# Autodesk Inventor assembly: Beamerscope_r2
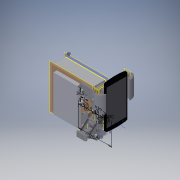
[picture p0: Inventor's stored thumbnail of the model, 180x180]
Saved by Autodesk Inventor 2016 (Build 200138000, 138)
## iProperties
Created: 2016-09-10
Part Number: Beamerscope_r2
Material: Generisch
Document SubType Name: Assembly
Designer: Bene
Mass: 220.683 g
Surface Area: 1737.49 cm^2
Volume: 289.423 cm^3
Density: 0.762493 g/cm^3
Author: Bene
## Documents named in this file (21)
- C:\Users\Bene\Dropbox\Dokumente\OpticalDesign\Beamerscope\Inventor\Beamerscope_r2\Beamerscope_r2.iam
- C:\Users\Bene\Dropbox\Dokumente\OpticalDesign\Beamerscope\Inventor\Beamerscope_r2\01_Beamer_Gehäuse.ipt
- C:\Users\Bene\Dropbox\Dokumente\OpticalDesign\Beamerscope\Inventor\Beamerscope_r2\02_Beamer_Deckel.ipt
- C:\Users\Bene\Dropbox\Dokumente\OpticalDesign\Beamerscope\Inventor\Beamerscope_r2\10_Mikrolinse.ipt
- C:\Users\Bene\Dropbox\Dokumente\OpticalDesign\Beamerscope\Inventor\Beamerscope_r2\11_Objektträger.ipt
- C:\Users\Bene\Dropbox\Dokumente\OpticalDesign\Beamerscope\Inventor\Beamerscope_r2\20_Z-Focus.ipt
- C:\Users\Bene\Dropbox\Dokumente\OpticalDesign\Beamerscope\Inventor\Beamerscope_r2\21_Connection_Projector_Focus.ipt
- C:\Users\Bene\Dropbox\Dokumente\OpticalDesign\Beamerscope\Inventor\Beamerscope_r2\31_Handyaufnahme_2.ipt
- C:\Users\Bene\Dropbox\Dokumente\OpticalDesign\Beamerscope\Inventor\Beamerscope_r2\31_Handyaufnahme_3.ipt
- C:\Users\Bene\Dropbox\Dokumente\OpticalDesign\Beamerscope\Inventor\Beamerscope_r2\00_SonyXperiaZ3correct.ipt
- C:\Users\Bene\Dropbox\Dokumente\OpticalDesign\Beamerscope\Inventor\Beamerscope_r2\32_Handycase.ipt
- C:\Users\Bene\Dropbox\Dokumente\OpticalDesign\Beamerscope\Inventor\Beamerscope_r2\22_Focus_Objectadapter.ipt
- C:\Users\Bene\Dropbox\Dokumente\OpticalDesign\Beamerscope\Inventor\Beamerscope_r2\31_Nexus 5.iam
- C:\Users\Bene\Dropbox\Dokumente\OpticalDesign\Beamerscope\Inventor\Beamerscope_r2\40_Adapter_Lens_Phone.ipt
- C:\Users\Bene\Dropbox\Dokumente\OpticalDesign\Beamerscope\Inventor\Beamerscope_r2\52_Bolzen.ipt
- C:\Users\Bene\Dropbox\Dokumente\OpticalDesign\Beamerscope\Inventor\Beamerscope_r2\22_Connection_Projector_Smartphone.ipt
- C:\Users\Bene\Dropbox\Dokumente\OpticalDesign\Beamerscope\Inventor\Beamerscope_r2\23_Connection_Smartphone.ipt
- C:\Users\Bene\Dropbox\Dokumente\OpticalDesign\Beamerscope\Inventor\Beamerscope_r2\00_Stange.ipt
- C:\Users\Bene\Dropbox\Dokumente\OpticalDesign\Beamerscope\Inventor\Beamerscope_r2\24_Klammer_rechts.ipt
- C:\Users\Bene\Dropbox\Dokumente\OpticalDesign\Beamerscope\Inventor\Beamerscope_r2\24_Klammer_links.ipt
- C:\Users\Bene\Dropbox\Dokumente\OpticalDesign\Beamerscope\Inventor\Beamerscope_r2\12_Lenstube.ipt
## Components (21 placed, 20 different names)
1. 01_Beamer_Gehäuse:1 — Fluchtend:1, Fluchtend:7, Fluchtend:8, Passend:6, Passend:7, Passend:8, Fluchtend:12, Fluchtend:13, Fluchtend:15, Fluchtend:24, Fluchtend:25, Passend:12
2. 02_Beamer_Deckel:1 — Fluchtend:1, Fluchtend:22
3. 10_Mikrolinse:1 — Passend:5
4. 11_Objektträger:1 — Passend:5
5. 20_Z-Focus:1 — Fluchtend:9, Fluchtend:11
6. 21_Connection_Projector_Focus:1 — Fluchtend:7, Fluchtend:8, Fluchtend:9
7. 31_Handyaufnahme_2:1 — Fluchtend:10, Einfügen:1, Einfügen:2, Passend:9, Winkel:2
8. 31_Handyaufnahme_3:1 — Passend:6, Passend:7, Passend:8, Passend:9, Winkel:2
9. 00_SonyXperiaZ3correct:1 — Fluchtend:10
10. 32_Handycase:1 — Einfügen:1, Einfügen:2
11. 22_Focus_Objectadapter:1 — Fluchtend:11, Fluchtend:23
12. 31_Nexus 5:1 [sub-assembly] — Passend:11
13. 40_Adapter_Lens_Phone:1 — Fluchtend:18
14. 52_Bolzen:1
15. 22_Connection_Projector_Smartphone:1 — Fluchtend:12, Fluchtend:13, Fluchtend:15, Fluchtend:16, Fluchtend:17
16. 23_Connection_Smartphone:1 — Fluchtend:16, Fluchtend:17, Fluchtend:18, Fluchtend:19, Passend:10, Fluchtend:21, Passend:11, Fluchtend:23
17. 00_Stange:1 — Fluchtend:19, Fluchtend:20
18. 00_Stange:2 — Passend:10, Fluchtend:20
19. 24_Klammer_rechts:1 — Fluchtend:21
20. 24_Klammer_links:1
21. 12_Lenstube:1 — Fluchtend:24, Fluchtend:25, Passend:12
## Relationships (30: Flush 19, Mate 8, Insert 2, Angle 1)
- Fluchtend:1 [Flush]: 01_Beamer_Gehäuse:1 ↔ 02_Beamer_Deckel:1
- Passend:5 [Mate]: 10_Mikrolinse:1 ↔ 11_Objektträger:1
- Fluchtend:7 [Flush]: 01_Beamer_Gehäuse:1 ↔ 21_Connection_Projector_Focus:1
- Fluchtend:8 [Flush]: 01_Beamer_Gehäuse:1 ↔ 21_Connection_Projector_Focus:1
- Fluchtend:9 [Flush]: 20_Z-Focus:1 ↔ 21_Connection_Projector_Focus:1
- Passend:6 [Mate]: 01_Beamer_Gehäuse:1 ↔ 31_Handyaufnahme_3:1
- Passend:7 [Mate]: 01_Beamer_Gehäuse:1 ↔ 31_Handyaufnahme_3:1
- Passend:8 [Mate]: 01_Beamer_Gehäuse:1 ↔ 31_Handyaufnahme_3:1
- Fluchtend:10 [Flush]: 31_Handyaufnahme_2:1 ↔ 00_SonyXperiaZ3correct:1
- Einfügen:1 [Insert] (-2 mm): 31_Handyaufnahme_2:1 ↔ 32_Handycase:1
- Einfügen:2 [Insert]: 31_Handyaufnahme_2:1 ↔ 32_Handycase:1
- Passend:9 [Mate]: 31_Handyaufnahme_2:1 ↔ 31_Handyaufnahme_3:1
- Fluchtend:11 [Flush]: 20_Z-Focus:1 ↔ 22_Focus_Objectadapter:1
- Winkel:2 [Angle] (0 deg): 31_Handyaufnahme_2:1 ↔ 31_Handyaufnahme_3:1
- Fluchtend:12 [Flush]: 01_Beamer_Gehäuse:1 ↔ 22_Connection_Projector_Smartphone:1
- Fluchtend:13 [Flush]: 01_Beamer_Gehäuse:1 ↔ 22_Connection_Projector_Smartphone:1
- Fluchtend:15 [Flush] (15 mm): 01_Beamer_Gehäuse:1 ↔ 22_Connection_Projector_Smartphone:1
- Fluchtend:16 [Flush]: 22_Connection_Projector_Smartphone:1 ↔ 23_Connection_Smartphone:1
- Fluchtend:17 [Flush]: 22_Connection_Projector_Smartphone:1 ↔ 23_Connection_Smartphone:1
- Fluchtend:18 [Flush]: 40_Adapter_Lens_Phone:1 ↔ 23_Connection_Smartphone:1
- Fluchtend:19 [Flush]: 23_Connection_Smartphone:1 ↔ 00_Stange:1
- Passend:10 [Mate]: 23_Connection_Smartphone:1 ↔ 00_Stange:2
- Fluchtend:20 [Flush]: 00_Stange:1 ↔ 00_Stange:2
- Fluchtend:21 [Flush]: 23_Connection_Smartphone:1 ↔ 24_Klammer_rechts:1
- Passend:11 [Mate]: 31_Nexus 5:1 ↔ 23_Connection_Smartphone:1
- Fluchtend:22 [Flush]: 02_Beamer_Deckel:1
- Fluchtend:23 [Flush] (-2 mm): 22_Focus_Objectadapter:1 ↔ 23_Connection_Smartphone:1
- Fluchtend:24 [Flush]: 01_Beamer_Gehäuse:1 ↔ 12_Lenstube:1
- Fluchtend:25 [Flush]: 01_Beamer_Gehäuse:1 ↔ 12_Lenstube:1
- Passend:12 [Mate]: 01_Beamer_Gehäuse:1 ↔ 12_Lenstube:1
